# Autodesk Inventor assembly: CyberDeckAssembly2
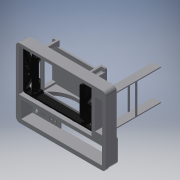
[picture p0: Inventor's stored thumbnail of the model, 180x180]
Saved by Autodesk Inventor 2019.4 (Build 234330000, 330)
## iProperties
Created: 2020-07-24
Part Number: CyberDeckAssembly2
Document SubType Name: Assembly
Designer: Briti
Author: Briti
## Documents named in this file (6)
- D:\3d prints\_MyModels\CyberDeck\CyberDeckAssembly2.iam
- D:\3d prints\_MyModels\CyberDeck\CyberDeckCover3.ipt
- D:\3d prints\_MyModels\Parts\servo-104.snapshot.1\Raspberry Pi Recovery Kit - Raspberry Pi Display Bracket.ipt
- D:\3d prints\_MyModels\CyberDeck\CyberDeckIOPanel2.ipt
- D:\3d prints\_MyModels\CyberDeck\CyberDeckVerticalInsert4.ipt
- D:\3d prints\_MyModels\CyberDeck\CyberDeckHDPower1.ipt
## Components (5 placed, 5 different names)
1. CyberDeckCover3:1 — Mate:1, Mate:2, Mate:3
2. Raspberry Pi Recovery Kit - Raspberry Pi Display Bracket:1 — Mate:1, Mate:4
3. CyberDeckIOPanel2:1 — Mate:2
4. CyberDeckVerticalInsert4:1 — Mate:3
5. CyberDeckHDPower1:1 — Mate:4
## Relationships (4: Mate 4)
- Mate:1: CyberDeckCover3:1 ↔ Raspberry Pi Recovery Kit - Raspberry Pi Display Bracket:1
- Mate:2: CyberDeckCover3:1 ↔ CyberDeckIOPanel2:1
- Mate:3: CyberDeckCover3:1 ↔ CyberDeckVerticalInsert4:1
- Mate:4: Raspberry Pi Recovery Kit - Raspberry Pi Display Bracket:1 ↔ CyberDeckHDPower1:1
